# Autodesk Inventor assembly: AssemblyGefreesdBase
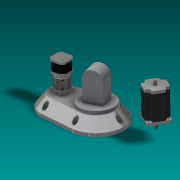
[picture p0: Inventor's stored thumbnail of the model, 180x180]
Saved by Autodesk Inventor 2020.2 (Build 242310000, 310)
## iProperties
Created: 2020-05-18
Part Number: AssemblyGefreesdBase
Document SubType Name: Assembly
Designer: Svend
Author: Svend
## Documents named in this file (15)
- C:\Users\Svend\OneDrive\Documents\GitHub\BeerMinder\3D-model\Base (Axis 1)\gefreesd\AssemblyGefreesdBase.iam
- C:\Users\Svend\OneDrive\Documents\GitHub\BeerMinder\3D-model\Base (Axis 1)\gefreesd\base bovenkant.ipt
- C:\Users\Svend\OneDrive\Documents\GitHub\BeerMinder\3D-model\bearings\51110 Groefkogellager - 70 mm.iam
- C:\Users\Svend\OneDrive\Documents\GitHub\BeerMinder\3D-model\subAssembly\Nema17MetGearbox.iam
- C:\Users\Svend\OneDrive\Documents\GitHub\BeerMinder\3D-model\gearbox\afstandsplaatje.ipt
- C:\Users\Svend\OneDrive\Documents\GitHub\BeerMinder\3D-model\bearings\Ball Bearing 608ZZ.ipt
- C:\Users\Svend\OneDrive\Documents\GitHub\BeerMinder\3D-model\Base (Axis 1)\gefreesd\onderkantBasegefreesd.ipt
- C:\Users\Svend\OneDrive\Documents\GitHub\BeerMinder\3D-model\pulleys\GT2 Timing Pulley 20T - 8mm as.ipt
- C:\Users\Svend\OneDrive\Documents\GitHub\BeerMinder\3D-model\pulleys\GT2 Timing Pulley 60T - 8mm as.ipt
- C:\Users\Svend\OneDrive\Documents\GitHub\BeerMinder\3D-model\pulleys\Tandriem20naar60T.ipt
- C:\Users\Svend\OneDrive\Documents\GitHub\BeerMinder\3D-model\Base (Axis 1)\AsBase.ipt
- C:\Users\Svend\OneDrive\Documents\Inventor\Content Center Files\R2020\en-US\ISO 14582_2013(E)\ISO 14582 - M5x20-10.9.ipt
- C:\Users\Svend\OneDrive\Documents\Inventor\Content Center Files\R2020\en-US\ISO 7380-1\ISO 7380-1 - M4 x 16.ipt
- C:\Users\Svend\OneDrive\Documents\GitHub\BeerMinder\3D-model\Base (Axis 1)\bevestiging axis 2.ipt
- C:\Users\Svend\OneDrive\Documents\GitHub\BeerMinder\3D-model\stepper motors\Nema 23 High toque.ipt
## Components (23 placed, 14 different names)
1. base bovenkant:1 — Mate:1, Mate:2, Mate:6, Mate:20, Mate:7, Flush:2, Mate:8, Mate:9, Mate:21, Mate:29, Mate:33, Mate:34, Mate:35, Mate:36, Mate:37
2. 51110 Groefkogellager - 70 mm:1 [sub-assembly] — Mate:1, Mate:2
3. Nema17MetGearbox:1 [sub-assembly] — Mate:3, Mate:4, Mate:5, Mate:20, Mate:13, Mate:28, Mate:30, Mate:31, Mate:32
4. afstandsplaatje:1 — Mate:3, Mate:4, Mate:5, Mate:6
5. Ball Bearing 608ZZ:1 — Mate:7, Flush:2, Mate:17
6. onderkantBasegefreesd:1 — Mate:8, Mate:9, Mate:10, Flush:3, Mate:18, Mate:21, Mate:22, Mate:23, Mate:24, Mate:25, Mate:26, Mate:27
7. GT2 Timing Pulley 20T - 8mm as:1 — Mate:13, Flush:4, Mate:15, Mate:16
8. GT2 Timing Pulley 60T - 8mm as:1 — Mate:11, Mate:12, Flush:4, Mate:14
9. Ball Bearing 608ZZ:2 — Mate:10, Flush:3, Mate:11, Mate:12
10. Tandriem20naar60T:1 — Mate:14, Mate:15, Mate:16
11. AsBase:1 — Mate:17, Mate:18
12. Screw ISO 14582:2013(E) M5x20-10.9:1 — Mate:22
13. Screw ISO 14582:2013(E) M5x20-10.9:6 — Mate:23
14. Screw ISO 14582:2013(E) M5x20-10.9:5 — Mate:24
15. Screw ISO 14582:2013(E) M5x20-10.9:4 — Mate:25
16. Screw ISO 14582:2013(E) M5x20-10.9:3 — Mate:26
17. Screw ISO 14582:2013(E) M5x20-10.9:2 — Mate:27
18. ISO 7380-1 M4 x 16:1 — Mate:28, Mate:29
19. ISO 7380-1 M4 x 16:2 — Mate:30, Mate:35
20. ISO 7380-1 M4 x 16:3 — Mate:32, Mate:34
21. ISO 7380-1 M4 x 16:4 — Mate:31, Mate:33
22. bevestiging axis 2:1 — Mate:36, Mate:37
23. Nema 23 High toque:1
## Relationships (39: Mate 36, Flush 3)
- Mate:1: base bovenkant:1 ↔ 51110 Groefkogellager - 70 mm:1
- Mate:2: base bovenkant:1 ↔ 51110 Groefkogellager - 70 mm:1
- Mate:3: Nema17MetGearbox:1 ↔ afstandsplaatje:1
- Mate:4: Nema17MetGearbox:1 ↔ afstandsplaatje:1
- Mate:5: Nema17MetGearbox:1 ↔ afstandsplaatje:1
- Mate:6: base bovenkant:1 ↔ afstandsplaatje:1
- Mate:20: base bovenkant:1 ↔ Nema17MetGearbox:1
- Mate:7: base bovenkant:1 ↔ Ball Bearing 608ZZ:1
- Flush:2: base bovenkant:1 ↔ Ball Bearing 608ZZ:1
- Mate:8: base bovenkant:1 ↔ onderkantBasegefreesd:1
- Mate:9: base bovenkant:1 ↔ onderkantBasegefreesd:1
- Mate:10: onderkantBasegefreesd:1 ↔ Ball Bearing 608ZZ:2
- Flush:3: onderkantBasegefreesd:1 ↔ Ball Bearing 608ZZ:2
- Mate:11: GT2 Timing Pulley 60T - 8mm as:1 ↔ Ball Bearing 608ZZ:2
- Mate:12: GT2 Timing Pulley 60T - 8mm as:1 ↔ Ball Bearing 608ZZ:2
- Mate:13: Nema17MetGearbox:1 ↔ GT2 Timing Pulley 20T - 8mm as:1
- Flush:4: GT2 Timing Pulley 20T - 8mm as:1 ↔ GT2 Timing Pulley 60T - 8mm as:1
- Mate:14: GT2 Timing Pulley 60T - 8mm as:1 ↔ Tandriem20naar60T:1
- Mate:15: GT2 Timing Pulley 20T - 8mm as:1 ↔ Tandriem20naar60T:1
- Mate:16 (0.5 mm): GT2 Timing Pulley 20T - 8mm as:1 ↔ Tandriem20naar60T:1
- Mate:17: Ball Bearing 608ZZ:1 ↔ AsBase:1
- Mate:18: onderkantBasegefreesd:1 ↔ AsBase:1
- Mate:21: base bovenkant:1 ↔ onderkantBasegefreesd:1
- Mate:22: onderkantBasegefreesd:1 ↔ Screw ISO 14582:2013(E) M5x20-10.9:1
- Mate:23: onderkantBasegefreesd:1 ↔ Screw ISO 14582:2013(E) M5x20-10.9:6
- Mate:24: onderkantBasegefreesd:1 ↔ Screw ISO 14582:2013(E) M5x20-10.9:5
- Mate:25: onderkantBasegefreesd:1 ↔ Screw ISO 14582:2013(E) M5x20-10.9:4
- Mate:26: onderkantBasegefreesd:1 ↔ Screw ISO 14582:2013(E) M5x20-10.9:3
- Mate:27: onderkantBasegefreesd:1 ↔ Screw ISO 14582:2013(E) M5x20-10.9:2
- Mate:28: Nema17MetGearbox:1 ↔ ISO 7380-1 M4 x 16:1
- Mate:29: base bovenkant:1 ↔ ISO 7380-1 M4 x 16:1
- Mate:30: Nema17MetGearbox:1 ↔ ISO 7380-1 M4 x 16:2
- Mate:31: Nema17MetGearbox:1 ↔ ISO 7380-1 M4 x 16:4
- Mate:32: Nema17MetGearbox:1 ↔ ISO 7380-1 M4 x 16:3
- Mate:33: base bovenkant:1 ↔ ISO 7380-1 M4 x 16:4
- Mate:34: base bovenkant:1 ↔ ISO 7380-1 M4 x 16:3
- Mate:35: base bovenkant:1 ↔ ISO 7380-1 M4 x 16:2
- Mate:36: base bovenkant:1 ↔ bevestiging axis 2:1
- Mate:37: base bovenkant:1 ↔ bevestiging axis 2:1
